# Autodesk Inventor assembly: fast_akkum2
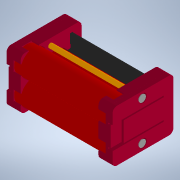
[picture p0: Inventor's stored thumbnail of the model, 180x180]
Saved by Autodesk Inventor 2020 (Build 240168000, 168)
## iProperties
Created: 2022-07-19
Part Number: fast_akkum2
Document SubType Name: Assembly
Designer: akapu
Author: akapu
## Documents named in this file (8)
- C:\Users\akapu\Documents\maze bot\fast_akkum2.iam
- C:\Users\akapu\Documents\maze bot\fast_battery_2.ipt
- C:\Users\akapu\Documents\maze bot\fast_battery.ipt
- C:\Users\akapu\Documents\maze bot\akkum_board.ipt
- C:\Users\akapu\Documents\maze bot\18650.ipt
- C:\Users\akapu\Documents\maze bot\fast_battery2_2.ipt
- C:\Users\akapu\Documents\maze bot\shelki.ipt
- C:\Users\akapu\Documents\maze bot\vint.ipt
## Components (9 placed, 7 different names)
1. fast_battery_2:1 — Жесткий:1, Вставка:1, Вставка:5
2. fast_battery:1 — Жесткий:1, Совмещение:1
3. akkum_board:1 — Совмещение:1
4. 18650:1 — Вставка:1, Вставка:2
5. fast_battery2_2:1 — Вставка:2, Вставка:4
6. shelki:1 — Вставка:4, С поворотом:1, С поворотом:2, Заподлицо:1
7. shelki:2 — Вставка:5
8. vint:1 — С поворотом:1
9. vint:2 — С поворотом:2, Заподлицо:1
## Relationships (9: Insert 4, RevoluteJoint 2, WeldJoint 1, Mate 1, Flush 1)
- Жесткий:1 [WeldJoint]: fast_battery_2:1 ↔ fast_battery:1
- Совмещение:1 [Mate]: fast_battery:1 ↔ akkum_board:1
- Вставка:1 [Insert] (-5 mm): fast_battery_2:1 ↔ 18650:1
- Вставка:2 [Insert]: 18650:1 ↔ fast_battery2_2:1
- Вставка:4 [Insert]: fast_battery2_2:1 ↔ shelki:1
- Вставка:5 [Insert]: fast_battery_2:1 ↔ shelki:2
- С поворотом:1 [RevoluteJoint]: shelki:1 ↔ vint:1
- С поворотом:2 [RevoluteJoint]: shelki:1 ↔ vint:2
- Заподлицо:1 [Flush]: shelki:1 ↔ vint:2
